# Autodesk Inventor assembly: plotter_new
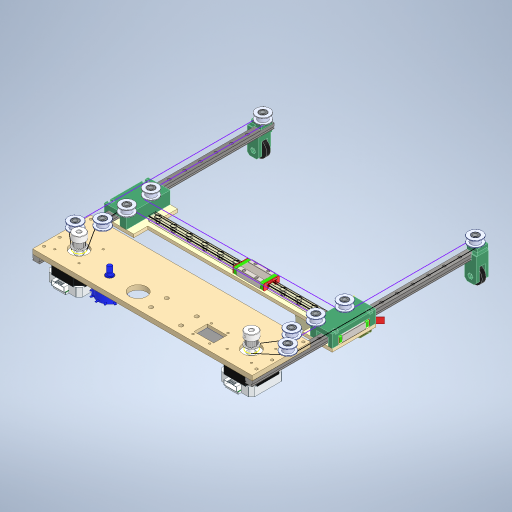
[picture p0: Inventor's stored thumbnail of the model, 512x512]
Saved by Autodesk Inventor 2023.1 (Build 271208000, 208)
## iProperties
Created: 2025-12-22
Part Number: plotter_new
Document SubType Name: Assembly
Designer: DELL
Author: DELL
## Documents named in this file (24)
- C:\Users\DELL\reposGitHub\VSOSH25-26\models\plotter\plotter_new.iam
- C:\Users\DELL\reposGitHub\VSOSH25-26\models\import\MGN9-H.ipt
- C:\Users\DELL\reposGitHub\VSOSH25-26\models\actuator\рельса.ipt
- C:\Users\DELL\reposGitHub\VSOSH25-26\models\import\Stepper motor Nema 17 (17HS2408).ipt
- C:\Users\DELL\reposGitHub\VSOSH25-26\models\actuator\центр_рейка.ipt
- C:\Users\DELL\reposGitHub\VSOSH25-26\models\actuator\креп_мотора.ipt
- C:\Users\DELL\reposGitHub\VSOSH25-26\models\import\Ролик с резьбой GT2 на моторы.ipt
- C:\Users\DELL\reposGitHub\VSOSH25-26\models\import\Сборка ролик с подшипником.ipt
- C:\Users\DELL\reposGitHub\VSOSH25-26\models\plotter\ограничитель.ipt
- C:\Users\DELL\reposGitHub\VSOSH25-26\models\actuator\рельса_центр.ipt
- C:\Users\DELL\reposGitHub\VSOSH25-26\models\import\Ролик с резьбой GT2 на моторы_MIR1.ipt
- C:\Users\DELL\reposGitHub\VSOSH25-26\models\import\Сборка ролик с подшипником_MIR3.ipt
- C:\Users\DELL\reposGitHub\VSOSH25-26\models\plotter\ограничитель_MIR.ipt
- C:\Users\DELL\reposGitHub\VSOSH25-26\models\actuator\креп_центр_м2.ipt
- C:\Users\DELL\reposGitHub\VSOSH25-26\models\import\Сборка ролик с подшипником_MIR4.ipt
- C:\Users\DELL\reposGitHub\VSOSH25-26\models\plotter\колесо.ipt
- C:\Users\DELL\reposGitHub\VSOSH25-26\models\import\RCL371-1-1-12.ipt
- C:\Users\DELL\reposGitHub\VSOSH25-26\models\plotter\концевик.ipt
- C:\Users\DELL\reposGitHub\VSOSH25-26\models\import\I2C OLED 128Ч64 Display Module.ipt
- C:\Users\DELL\reposGitHub\VSOSH25-26\models\import\TCRT5000.ipt
- C:\Users\DELL\reposGitHub\VSOSH25-26\models\plotter\креп_опт.ipt
- C:\Users\DELL\reposGitHub\VSOSH25-26\models\plotter\креп_концевика.ipt
- C:\Users\DELL\reposGitHub\VSOSH25-26\models\actuator\креп_центр_м2_MIR1.ipt
- C:\Users\DELL\reposGitHub\VSOSH25-26\models\plotter\ремень.ipt
## Components (35 placed, 23 different names)
1. рельса:1 — Совмещение:1, Совмещение:11, Заподлицо:7, Совмещение:12, Заподлицо:9, Совмещение:62, Совмещение:63, Совмещение:90, Совмещение:91, Заподлицо:25, Совмещение:106
2. Stepper motor Nema 17 (17HS2408):2 — Заподлицо:7, Совмещение:12, Заподлицо:18, Совмещение:18, Заподлицо:25
3. рельса:2 — Заподлицо:13, Заподлицо:15, Совмещение:15, Совмещение:16, Заподлицо:16, Совмещение:50, Совмещение:51, Заподлицо:26, Совмещение:107
4. MGN9-H:2 — Совмещение:49
5. Stepper motor Nema 17 (17HS2408):3 — Заподлицо:15, Совмещение:15, Совмещение:60, Заподлицо:26
6. креп_мотора:1 — Заподлицо:18, Совмещение:19, Совмещение:94, Совмещение:95, Совмещение:96, Совмещение:97, Совмещение:98, Совмещение:99, Совмещение:100, Совмещение:101, Касательность:2, Совмещение:113, Совмещение:114, Совмещение:115, Совмещение:116, Совмещение:117
7. Ролик с резьбой GT2 на моторы:1 — Совмещение:18, Совмещение:19
8. Сборка ролик с подшипником:1 — Совмещение:94, Совмещение:95
9. ограничитель:1 — Совмещение:90, Совмещение:91, Совмещение:92, Совмещение:93, Совмещение:102, Совмещение:103, Совмещение:106
10. Сборка ролик с подшипником:2 — Совмещение:92, Совмещение:93
11. Сборка ролик с подшипником:4 — Совмещение:160, Совмещение:161
12. Сборка ролик с подшипником:5 — Совмещение:162, Совмещение:166
13. рельса_центр:1 — Совмещение:37, Совмещение:38, Совмещение:52, Заподлицо:23, Совмещение:154
14. MGN9-H:3 — Совмещение:37, Совмещение:38
15. Ролик с резьбой GT2 на моторы_MIR1:1 — Совмещение:60
16. ограничитель_MIR:1 — Совмещение:39, Совмещение:40, Совмещение:50, Совмещение:51, Совмещение:104, Совмещение:105, Совмещение:107
17. Сборка ролик с подшипником_MIR3:2 — Совмещение:39, Совмещение:40
18. центр_рейка:1 — Совмещение:49, Совмещение:52, Заподлицо:23, Совмещение:66, Совмещение:67, Совмещение:127, Совмещение:136, Совмещение:145, Совмещение:146, Совмещение:147, Совмещение:148, Совмещение:149, Совмещение:155, Совмещение:156, Совмещение:157, Совмещение:158, Совмещение:163, Совмещение:164
19. MGN9-H:4 — Совмещение:62, Совмещение:63, Совмещение:66, Совмещение:67, Совмещение:127
20. Сборка ролик с подшипником_MIR4:1 — Совмещение:150, Совмещение:153
21. Сборка ролик с подшипником_MIR4:2 — Совмещение:152, Совмещение:165
22. Сборка ролик с подшипником:6 — Совмещение:96, Совмещение:97
23. Сборка ролик с подшипником:7 — Совмещение:98, Совмещение:99
24. Сборка ролик с подшипником:8 — Совмещение:100, Совмещение:101
25. колесо:1 — Совмещение:102, Совмещение:103
26. колесо:2 — Совмещение:104, Совмещение:105
27. RCL371-1-1-12:1 — Касательность:2, Совмещение:113, Совмещение:114
28. концевик:1 — Совмещение:133, Совмещение:134, Совмещение:135
29. I2C OLED 128Ч64 Display Module:1 — Совмещение:115, Совмещение:116, Совмещение:117
30. креп_центр_м2:1 — Совмещение:147, Совмещение:148, Совмещение:149, Совмещение:150, Совмещение:152, Совмещение:153, Совмещение:154, Совмещение:165
31. креп_концевика:2 — Совмещение:133, Совмещение:134, Совмещение:135, Совмещение:136, Совмещение:146, Совмещение:155
32. TCRT5000:1 — Совмещение:142, Совмещение:143, Совмещение:144
33. креп_опт:1 — Совмещение:142, Совмещение:143, Совмещение:144, Совмещение:145, Совмещение:163, Совмещение:164
34. креп_центр_м2_MIR1:1 — Совмещение:156, Совмещение:157, Совмещение:158, Совмещение:160, Совмещение:161, Совмещение:162, Совмещение:166, Заподлицо:27
35. ремень:1 — Заподлицо:27
## Relationships (84: Mate 73, Flush 10, Tangent 1)
- Совмещение:1 [Mate] (131.4 mm): рельса:1
- Совмещение:11 [Mate]: рельса:1
- Заподлицо:7 [Flush]: рельса:1 ↔ Stepper motor Nema 17 (17HS2408):2
- Совмещение:12 [Mate]: рельса:1 ↔ Stepper motor Nema 17 (17HS2408):2
- Заподлицо:9 [Flush] (150 mm): рельса:1
- [Mate]: рельса:2 ↔ MGN9-H:2
- [Mate] (-0.2 mm): рельса:2 ↔ MGN9-H:2
- Заподлицо:13 [Flush] (-150 mm): рельса:2
- Заподлицо:15 [Flush]: рельса:2 ↔ Stepper motor Nema 17 (17HS2408):3
- Совмещение:15 [Mate]: рельса:2 ↔ Stepper motor Nema 17 (17HS2408):3
- Совмещение:16 [Mate]: рельса:2
- Заподлицо:16 [Flush] (131.4 mm): рельса:2
- Заподлицо:18 [Flush]: Stepper motor Nema 17 (17HS2408):2 ↔ креп_мотора:1
- Совмещение:18 [Mate]: Stepper motor Nema 17 (17HS2408):2 ↔ Ролик с резьбой GT2 на моторы:1
- Совмещение:19 [Mate] (5 mm): креп_мотора:1 ↔ Ролик с резьбой GT2 на моторы:1
- Совмещение:37 [Mate]: рельса_центр:1 ↔ MGN9-H:3
- Совмещение:38 [Mate] (0.2 mm): рельса_центр:1 ↔ MGN9-H:3
- Совмещение:39 [Mate]: ограничитель_MIR:1 ↔ Сборка ролик с подшипником_MIR3:2
- Совмещение:40 [Mate]: ограничитель_MIR:1 ↔ Сборка ролик с подшипником_MIR3:2
- Совмещение:49 [Mate]: MGN9-H:2 ↔ центр_рейка:1
- Совмещение:50 [Mate]: рельса:2 ↔ ограничитель_MIR:1
- Совмещение:51 [Mate]: рельса:2 ↔ ограничитель_MIR:1
- Совмещение:52 [Mate]: рельса_центр:1 ↔ центр_рейка:1
- Заподлицо:23 [Flush] (-23.5 mm): рельса_центр:1 ↔ центр_рейка:1
- Совмещение:60 [Mate]: Stepper motor Nema 17 (17HS2408):3 ↔ Ролик с резьбой GT2 на моторы_MIR1:1
- Совмещение:62 [Mate]: рельса:1 ↔ MGN9-H:4
- Совмещение:63 [Mate] (-0.2 mm): рельса:1 ↔ MGN9-H:4
- Совмещение:66 [Mate]: центр_рейка:1 ↔ MGN9-H:4
- Совмещение:67 [Mate]: центр_рейка:1 ↔ MGN9-H:4
- Совмещение:90 [Mate]: рельса:1 ↔ ограничитель:1
- Совмещение:91 [Mate]: рельса:1 ↔ ограничитель:1
- Совмещение:92 [Mate]: ограничитель:1 ↔ Сборка ролик с подшипником:2
- Совмещение:93 [Mate]: ограничитель:1 ↔ Сборка ролик с подшипником:2
- Заподлицо:25 [Flush] (8 mm): рельса:1 ↔ Stepper motor Nema 17 (17HS2408):2
- Заподлицо:26 [Flush] (-8 mm): рельса:2 ↔ Stepper motor Nema 17 (17HS2408):3
- Совмещение:94 [Mate]: креп_мотора:1 ↔ Сборка ролик с подшипником:1
- Совмещение:95 [Mate]: креп_мотора:1 ↔ Сборка ролик с подшипником:1
- Совмещение:96 [Mate]: креп_мотора:1 ↔ Сборка ролик с подшипником:6
- Совмещение:97 [Mate]: креп_мотора:1 ↔ Сборка ролик с подшипником:6
- Совмещение:98 [Mate]: креп_мотора:1 ↔ Сборка ролик с подшипником:7
- Совмещение:99 [Mate]: креп_мотора:1 ↔ Сборка ролик с подшипником:7
- Совмещение:100 [Mate]: креп_мотора:1 ↔ Сборка ролик с подшипником:8
- Совмещение:101 [Mate]: креп_мотора:1 ↔ Сборка ролик с подшипником:8
- Совмещение:102 [Mate]: ограничитель:1 ↔ колесо:1
- Совмещение:103 [Mate]: ограничитель:1 ↔ колесо:1
- Совмещение:104 [Mate]: ограничитель_MIR:1 ↔ колесо:2
- Совмещение:105 [Mate]: ограничитель_MIR:1 ↔ колесо:2
- Совмещение:106 [Mate] (0.2 mm): рельса:1 ↔ ограничитель:1
- Совмещение:107 [Mate] (0.2 mm): рельса:2 ↔ ограничитель_MIR:1
- Касательность:2 [Tangent] (-90 mm): креп_мотора:1 ↔ RCL371-1-1-12:1
- Совмещение:113 [Mate]: креп_мотора:1 ↔ RCL371-1-1-12:1
- Совмещение:114 [Mate]: креп_мотора:1 ↔ RCL371-1-1-12:1
- Совмещение:115 [Mate]: креп_мотора:1 ↔ I2C OLED 128Ч64 Display Module:1
- Совмещение:116 [Mate]: креп_мотора:1 ↔ I2C OLED 128Ч64 Display Module:1
- Совмещение:117 [Mate]: креп_мотора:1 ↔ I2C OLED 128Ч64 Display Module:1
- Совмещение:127 [Mate]: центр_рейка:1 ↔ MGN9-H:4
- Совмещение:133 [Mate]: концевик:1 ↔ креп_концевика:2
- Совмещение:134 [Mate]: концевик:1 ↔ креп_концевика:2
- Совмещение:135 [Mate]: концевик:1 ↔ креп_концевика:2
- Совмещение:136 [Mate]: центр_рейка:1 ↔ креп_концевика:2
- Совмещение:142 [Mate]: TCRT5000:1 ↔ креп_опт:1
- Совмещение:143 [Mate]: TCRT5000:1 ↔ креп_опт:1
- Совмещение:144 [Mate]: TCRT5000:1 ↔ креп_опт:1
- Совмещение:145 [Mate]: центр_рейка:1 ↔ креп_опт:1
- Совмещение:146 [Mate]: центр_рейка:1 ↔ креп_концевика:2
- Совмещение:147 [Mate]: центр_рейка:1 ↔ креп_центр_м2:1
- Совмещение:148 [Mate]: центр_рейка:1 ↔ креп_центр_м2:1
- Совмещение:149 [Mate]: центр_рейка:1 ↔ креп_центр_м2:1
- Совмещение:150 [Mate]: Сборка ролик с подшипником_MIR4:1 ↔ креп_центр_м2:1
- Совмещение:152 [Mate]: Сборка ролик с подшипником_MIR4:2 ↔ креп_центр_м2:1
- Совмещение:153 [Mate]: Сборка ролик с подшипником_MIR4:1 ↔ креп_центр_м2:1
- Совмещение:154 [Mate] (5 mm): рельса_центр:1 ↔ креп_центр_м2:1
- Совмещение:155 [Mate]: центр_рейка:1 ↔ креп_концевика:2
- Совмещение:156 [Mate]: центр_рейка:1 ↔ креп_центр_м2_MIR1:1
- Совмещение:157 [Mate]: центр_рейка:1 ↔ креп_центр_м2_MIR1:1
- Совмещение:158 [Mate]: центр_рейка:1 ↔ креп_центр_м2_MIR1:1
- Совмещение:160 [Mate]: Сборка ролик с подшипником:4 ↔ креп_центр_м2_MIR1:1
- Совмещение:161 [Mate]: Сборка ролик с подшипником:4 ↔ креп_центр_м2_MIR1:1
- Совмещение:162 [Mate]: Сборка ролик с подшипником:5 ↔ креп_центр_м2_MIR1:1
- Совмещение:163 [Mate]: центр_рейка:1 ↔ креп_опт:1
- Совмещение:164 [Mate]: центр_рейка:1 ↔ креп_опт:1
- Совмещение:165 [Mate]: Сборка ролик с подшипником_MIR4:2 ↔ креп_центр_м2:1
- Совмещение:166 [Mate]: Сборка ролик с подшипником:5 ↔ креп_центр_м2_MIR1:1
- Заподлицо:27 [Flush]: креп_центр_м2_MIR1:1 ↔ ремень:1
## Named parameters: d34_d9 = 0 mm, d35_d10 = -0.2 mm
